# Autodesk Inventor assembly: kamera gesamt
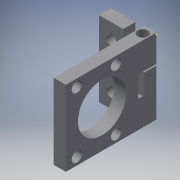
[picture p0: Inventor's stored thumbnail of the model, 180x180]
Saved by Autodesk Inventor 2018 (Build 220112000, 112)
## iProperties
Created: 2018-01-30
Part Number: kamera gesamt
Material: Generisch
Document SubType Name: Assembly
Designer: Andreas
Author: Andreas
## Documents named in this file (3)
- C:\Users\Andreas\Desktop\Anna\SPS\Embedded Systems\kamera gesamt.iam
- C:\Users\Andreas\Desktop\Anna\SPS\Embedded Systems\kamera ot.ipt
- C:\Users\Andreas\Desktop\Anna\SPS\Embedded Systems\kamera ut.ipt
## Components (2 placed, 2 different names)
1. kamera ot:1 — Drehbar:1, Drehbar:2, Drehbar:3, Drehbar:4
2. kamera ut:1 — Drehbar:1, Drehbar:2, Drehbar:3, Drehbar:4
## Relationships (4: RevoluteJoint 4)
- Drehbar:1 [RevoluteJoint] (45 mm): kamera ot:1 ↔ kamera ut:1
- Drehbar:2 [RevoluteJoint]: kamera ot:1 ↔ kamera ut:1
- Drehbar:3 [RevoluteJoint]: kamera ot:1 ↔ kamera ut:1
- Drehbar:4 [RevoluteJoint]: kamera ot:1 ↔ kamera ut:1
